# Autodesk Inventor assembly: Bolt outline
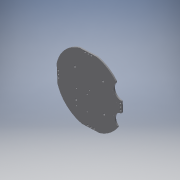
[picture p0: Inventor's stored thumbnail of the model, 180x180]
Saved by Autodesk Inventor 2017 (Build 210142000, 142)
## iProperties
Created: 2017-03-28
Part Number: Bolt outline
Document SubType Name: Assembly
Designer: qupec
Author: qupec
## Documents named in this file (3)
- D:\UMD Near Space\STAR\CAD\Mechanical\CapTech\Bolt outline.iam
- D:\UMD Near Space\STAR\CAD\Mechanical\CapTech\RSX Deck.ipt
- D:\UMD Near Space\STAR\CAD\Mechanical\Base Plate Mk 2.ipt
## Components (2 placed, 2 different names)
1. RSX Deck:1 — Mate:1, Mate:2, Mate:3
2. Base Plate Mk 2:1 — Mate:1, Mate:2, Mate:3
## Relationships (3: Mate 3)
- Mate:1: RSX Deck:1 ↔ Base Plate Mk 2:1
- Mate:2: RSX Deck:1 ↔ Base Plate Mk 2:1
- Mate:3: RSX Deck:1 ↔ Base Plate Mk 2:1
